# Autodesk Inventor assembly: 05_birdeyeArm
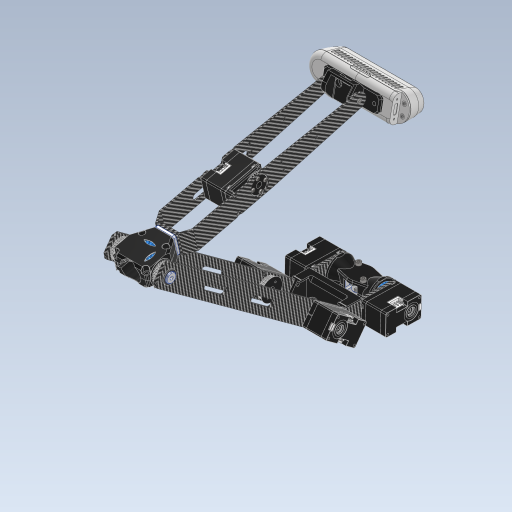
[picture p0: Inventor's stored thumbnail of the model, 512x512]
Saved by Autodesk Inventor 2024 (Build 280153000, 153)
## iProperties
Created: 2023-09-03
Part Number: 05_birdeyeArm
Document SubType Name: Assembly
Designer: michi
Mass: 322.253 g
Surface Area: 2683.15 cm^2
Volume: 262.932 cm^3
Density: 1.22562 g/cm^3
Author: michi
## Documents named in this file (14)
- C:\Users\michi\OneDrive\default\robotis\DynamixelExamples\DynamixelXC330MiniArm\CAD_inventor\05_birdeye.iam
- C:\Users\michi\OneDrive\default\robotis\DynamixelExamples\DynamixelXC330MiniArm\CAD_inventor\_bridseye_sketch.ipt
- C:\Users\michi\OneDrive\default\robotis\DynamixelExamples\DynamixelXC330MiniArm\CAD_inventor\brideye_links\brideye_links_link1.ipt
- C:\Users\michi\OneDrive\default\robotis\DynamixelExamples\DynamixelXC330MiniArm\CAD_inventor\brideye_links\brideye_links_link1_MIR.ipt
- C:\Users\michi\OneDrive\default\robotis\DynamixelExamples\DynamixelXC330MiniArm\CAD_inventor\birdeye_shoulderUnit.iam
- C:\Users\michi\OneDrive\default\robotis\DynamixelExamples\DynamixelXC330MiniArm\CAD_inventor\birdeye__screw\Bolt_M2_10mm-selfTap_CSPPNSB-STU-TP2-10_203.ipt
- C:\Users\michi\OneDrive\default\robotis\DynamixelExamples\DynamixelXC330MiniArm\CAD_inventor\brideye_links\brideye_links_link1Conn.ipt
- C:\Users\michi\OneDrive\default\robotis\DynamixelExamples\DynamixelXC330MiniArm\CAD_inventor\birdeye_elbowUnit\birdeye_elbowUnit_actuator.iam
- C:\Users\michi\OneDrive\default\robotis\DynamixelExamples\DynamixelXC330MiniArm\CAD_inventor\birdeye_elbowUnit.iam
- C:\Users\michi\OneDrive\default\robotis\DynamixelExamples\DynamixelXC330MiniArm\CAD_inventor\birdeye_wristUnit.iam
- C:\Users\michi\OneDrive\default\robotis\DynamixelExamples\DynamixelXC330MiniArm\CAD_inventor\brideye_links\brideye_links_link2_Left.ipt
- C:\Users\michi\OneDrive\default\robotis\DynamixelExamples\DynamixelXC330MiniArm\CAD_inventor\brideye_links\brideye_links_link2_Right.ipt
- C:\Users\michi\OneDrive\default\robotis\DynamixelExamples\DynamixelXC330MiniArm\CAD_inventor\birdeye_wristUnit\birdeye_wristUnit_actuator.iam
- C:\Users\michi\OneDrive\default\robotis\DynamixelExamples\DynamixelXC330MiniArm\CAD_inventor\birdeye_wristUnit\realsense.iam
## Components (15 placed, 13 different names)
1. _bridseye_sketch:1
2. brideye_links_link1:1 — 回転:1, 回転:2, 回転:13
3. brideye_links_link1_MIR:1 — 回転:3, 回転:4, 回転:5, 回転:14, 回転:29, 回転:30, メイト:3
4. birdeye_shoulderUnit:1 [sub-assembly] — 回転:1, 回転:2, 回転:3, 回転:4
5. Bolt_M2_10mm-selfTap_CSPPNSB-STU-TP2-10_203:1 — 回転:5
6. brideye_links_link1Conn:1 — 回転:13, メイト:3
7. birdeye_elbowUnit_actuator:1 [sub-assembly]
8. birdeye_elbowUnit_actuator:2 [sub-assembly] — 回転:29, 回転:30
9. birdeye_elbowUnit:1 [sub-assembly] — 回転:14, 回転:31, 回転:32
10. birdeye_wristUnit:1 [sub-assembly] — 回転:37, 回転:39, 回転:40
11. brideye_links_link2_Left:1 — 回転:31, 回転:32, 回転:33, 回転:34, 回転:35, 回転:36, 回転:37, 回転:38
12. brideye_links_link2_Right:1 — 回転:33, 回転:34
13. birdeye_wristUnit_actuator:1 [sub-assembly] — 回転:35, 回転:36
14. Bolt_M2_10mm-selfTap_CSPPNSB-STU-TP2-10_203:2 — 回転:38
15. realsense:1 [sub-assembly] — 回転:39, 回転:40
## Relationships (22: RevoluteJoint 21, Mate 1)
- 回転:1 [RevoluteJoint]: brideye_links_link1:1 ↔ birdeye_shoulderUnit:1
- 回転:2 [RevoluteJoint]: brideye_links_link1:1 ↔ birdeye_shoulderUnit:1
- 回転:3 [RevoluteJoint]: brideye_links_link1_MIR:1 ↔ birdeye_shoulderUnit:1
- 回転:4 [RevoluteJoint]: brideye_links_link1_MIR:1 ↔ birdeye_shoulderUnit:1
- 回転:5 [RevoluteJoint]: brideye_links_link1_MIR:1 ↔ Bolt_M2_10mm-selfTap_CSPPNSB-STU-TP2-10_203:1
- [RevoluteJoint]: brideye_links_link1:1 ↔ birdeye_elbowUnit_actuator:1
- [RevoluteJoint]: brideye_links_link1:1 ↔ birdeye_elbowUnit_actuator:1
- 回転:13 [RevoluteJoint]: brideye_links_link1:1 ↔ brideye_links_link1Conn:1
- 回転:14 [RevoluteJoint]: brideye_links_link1_MIR:1 ↔ birdeye_elbowUnit:1
- 回転:29 [RevoluteJoint]: brideye_links_link1_MIR:1 ↔ birdeye_elbowUnit_actuator:2
- 回転:30 [RevoluteJoint]: brideye_links_link1_MIR:1 ↔ birdeye_elbowUnit_actuator:2
- 回転:31 [RevoluteJoint]: birdeye_elbowUnit:1 ↔ brideye_links_link2_Left:1
- 回転:32 [RevoluteJoint]: birdeye_elbowUnit:1 ↔ brideye_links_link2_Left:1
- 回転:33 [RevoluteJoint]: brideye_links_link2_Left:1 ↔ brideye_links_link2_Right:1
- 回転:34 [RevoluteJoint]: brideye_links_link2_Left:1 ↔ brideye_links_link2_Right:1
- 回転:35 [RevoluteJoint]: brideye_links_link2_Left:1 ↔ birdeye_wristUnit_actuator:1
- 回転:36 [RevoluteJoint]: brideye_links_link2_Left:1 ↔ birdeye_wristUnit_actuator:1
- メイト:3 [Mate]: brideye_links_link1_MIR:1 ↔ brideye_links_link1Conn:1
- 回転:37 [RevoluteJoint]: birdeye_wristUnit:1 ↔ brideye_links_link2_Left:1
- 回転:38 [RevoluteJoint]: brideye_links_link2_Left:1 ↔ Bolt_M2_10mm-selfTap_CSPPNSB-STU-TP2-10_203:2
- 回転:39 [RevoluteJoint]: birdeye_wristUnit:1 ↔ realsense:1
- 回転:40 [RevoluteJoint]: birdeye_wristUnit:1 ↔ realsense:1
